# Autodesk Inventor assembly: Arm
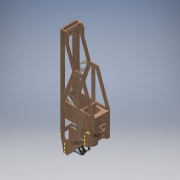
[picture p0: Inventor's stored thumbnail of the model, 180x180]
Saved by Autodesk Inventor 2019 (Build 230136000, 136)
## iProperties
Created: 2019-01-14
Part Number: Arm
Document SubType Name: Assembly
Designer: nxgam
Mass: 1682.66 g
Surface Area: 7952.13 cm^2
Volume: 1677.12 cm^3
Density: 1.0033 g/cm^3
Author: nxgam
## Documents named in this file (20)
- C:\Users\nxgam\Documents\CAD\Inventor\DiscoDraw\Arm.iam
- C:\Users\nxgam\Documents\CAD\Inventor\DiscoDraw\Arm.ipt
- C:\Users\nxgam\Documents\CAD\Inventor\DiscoDraw\Sled.iam
- C:\Users\nxgam\Documents\CAD\Inventor\DiscoDraw\ArmSpacer.ipt
- C:\Users\nxgam\Documents\CAD\Inventor\DiscoDraw\ArmSpacer3.ipt
- C:\Users\nxgam\Documents\CAD\Inventor\DiscoDraw\ArmSpacer6.ipt
- C:\Users\nxgam\Documents\CAD\Inventor\DiscoDraw\ArmTo.ipt
- C:\Users\nxgam\Documents\CAD\Inventor\DiscoDraw\ArmSide.ipt
- C:\Users\nxgam\Documents\CAD\Inventor\DiscoDraw\ArmMount.ipt
- C:\Users\nxgam\Documents\CAD\Inventor\DiscoDraw\MotorShelf.ipt
- C:\Users\nxgam\Documents\CAD\Inventor\DiscoDraw\EndPulleyMount.ipt
- C:\Users\nxgam\Documents\CAD\Inventor\DiscoDraw\ArmSideFrong2.ipt
- C:\Users\nxgam\Documents\CAD\Inventor\DiscoDraw\PiShelf.iam
- C:\Users\nxgam\Documents\CAD\Inventor\DiscoDraw\VerticalSupport.ipt
- C:\Users\nxgam\Documents\CAD\Inventor\DiscoDraw\LimitSwitch.ipt
- C:\Users\nxgam\Documents\CAD\Inventor\DiscoDraw\LimitSwitchMount.ipt
- C:\Users\nxgam\Documents\CAD\Inventor\DiscoDraw\BearingMount.ipt
- C:\Users\nxgam\Documents\CAD\Inventor\DiscoDraw\Imported\DC Motor\Motor assembly.ipt
- C:\Users\nxgam\Documents\CAD\Inventor\DiscoDraw\MotorMountDC.ipt
- C:\Users\nxgam\Documents\CAD\Inventor\DiscoDraw\MotorMountDCB.ipt
## Components (28 placed, 19 different names)
1. Arm:1 — Mate:1, Angle:1, Mate:4, Mate:5, Mate:6, Flush:3, Flush:4, Mate:7, Flush:12, Flush:13
2. Sled:1 [sub-assembly] — Mate:1, Angle:1, Flush:2, Flush:59
3. ArmSpacer:1 — Mate:3, Mate:5, Flush:1, Flush:4, Flush:10, Flush:11, Mate:8
4. ArmSpacer:2 — Mate:3, Mate:4, Flush:1, Flush:3
5. ArmSpacer3:1 — Flush:7, Mate:7, Flush:9
6. ArmSpacer3:3 — Flush:5, Flush:8
7. ArmSpacer6:1 — Flush:5, Flush:6, Flush:8, Flush:11
8. ArmSpacer6:2 — Flush:6, Flush:7, Flush:9, Flush:10
9. ArmTo:1 — Flush:12, Flush:13, Mate:8, Flush:28, Flush:29, Flush:31, Mate:20, Flush:54, Flush:57, Mate:31, Mate:32
10. ArmSide:1 — Flush:23, Flush:25, Flush:31, Flush:35, Flush:36, Flush:37, Mate:13, Mate:19, Flush:43, Flush:50, Mate:23, Flush:51, Mate:27, Mate:39
11. ArmSide:2 — Flush:26, Flush:27, Flush:28, Flush:29, Mate:15, Flush:46, Flush:49, Mate:21, Flush:50, Mate:24, Flush:55, Flush:56, Mate:30, Mate:37
12. ArmMount:1 — Flush:20, Flush:21, Flush:23, Flush:25, Flush:26, Flush:27, Mate:27, Mate:34, Mate:35, Angle:2
13. ArmMount:2 — Flush:20, Flush:21, Mate:28
14. VerticalSupport:2 — Flush:35, Flush:38, Mate:13
15. VerticalSupport:1 — Flush:36, Flush:37, Flush:38, Mate:15, Mate:36, Flush:61, Angle:3, Mate:42
16. EndPulleyMount:1 — Mate:19, Mate:20, Flush:53
17. ArmSideFrong2:1 — Flush:43, Flush:47, Flush:48, Mate:25, Flush:52, Mate:26, Flush:53, Flush:54, Mate:28
18. ArmSideFrong2:2 — Flush:46, Flush:47, Flush:48, Flush:49, Mate:21
19. PiShelf:1 [sub-assembly] — Flush:55, Flush:56, Mate:30
20. MotorShelf:1 — Mate:25, Flush:52, Mate:26
21. MotorShelf:2 — Mate:23, Mate:24, Flush:51
22. LimitSwitch:1 — Flush:57, Mate:31, Mate:33, Flush:58, Flush:60
23. LimitSwitchMount:1 — Mate:32, Mate:33, Flush:58
24. BearingMount:1 — Mate:34, Mate:35, Angle:2
25. Motor assembly:1 — Angle:3, Mate:41, Mate:42
26. MotorMountDC:1 — Mate:36, Flush:61, Mate:37, Mate:38, Flush:62
27. MotorMountDC:3
28. MotorMountDCB:1 — Mate:38, Flush:62, Mate:39, Mate:41
## Relationships (77: Flush 44, Mate 30, Angle 3)
- Mate:1: Arm:1 ↔ Sled:1
- Angle:1 (0 deg): Arm:1 ↔ Sled:1
- Mate:3: ArmSpacer:1 ↔ ArmSpacer:2
- Mate:4: Arm:1 ↔ ArmSpacer:2
- Mate:5: Arm:1 ↔ ArmSpacer:1
- Flush:1: ArmSpacer:1 ↔ ArmSpacer:2
- Flush:2 (-2.54 mm): Sled:1
- Mate:6: Arm:1
- Flush:3: Arm:1 ↔ ArmSpacer:2
- Flush:4: Arm:1 ↔ ArmSpacer:1
- Flush:5: ArmSpacer3:3 ↔ ArmSpacer6:1
- Flush:6: ArmSpacer6:1 ↔ ArmSpacer6:2
- Flush:7: ArmSpacer3:1 ↔ ArmSpacer6:2
- Mate:7: Arm:1 ↔ ArmSpacer3:1
- Flush:8: ArmSpacer3:3 ↔ ArmSpacer6:1
- Flush:9: ArmSpacer3:1 ↔ ArmSpacer6:2
- Flush:10: ArmSpacer:1 ↔ ArmSpacer6:2
- Flush:11: ArmSpacer:1 ↔ ArmSpacer6:1
- Flush:12: Arm:1 ↔ ArmTo:1
- Flush:13: Arm:1 ↔ ArmTo:1
- Mate:8: ArmSpacer:1 ↔ ArmTo:1
- Flush:20: ArmMount:1 ↔ ArmMount:2
- Flush:21: ArmMount:1 ↔ ArmMount:2
- Flush:23: ArmSide:1 ↔ ArmMount:1
- Flush:25: ArmSide:1 ↔ ArmMount:1
- Flush:26: ArmSide:2 ↔ ArmMount:1
- Flush:27: ArmSide:2 ↔ ArmMount:1
- Flush:28: ArmTo:1 ↔ ArmSide:2
- Flush:29: ArmTo:1 ↔ ArmSide:2
- Flush:31: ArmTo:1 ↔ ArmSide:1
- Flush:35: ArmSide:1 ↔ VerticalSupport:2
- Flush:36: ArmSide:1 ↔ VerticalSupport:1
- Flush:37: ArmSide:1 ↔ VerticalSupport:1
- Flush:38: VerticalSupport:2 ↔ VerticalSupport:1
- Mate:13: ArmSide:1 ↔ VerticalSupport:2
- Mate:15: ArmSide:2 ↔ VerticalSupport:1
- Mate:19: ArmSide:1 ↔ EndPulleyMount:1
- Mate:20 (20.32 mm): ArmTo:1 ↔ EndPulleyMount:1
- Flush:43: ArmSide:1 ↔ ArmSideFrong2:1
- Flush:46: ArmSide:2 ↔ ArmSideFrong2:2
- Flush:47: ArmSideFrong2:1 ↔ ArmSideFrong2:2
- Flush:48: ArmSideFrong2:1 ↔ ArmSideFrong2:2
- Flush:49: ArmSide:2 ↔ ArmSideFrong2:2
- Mate:21: ArmSide:2 ↔ ArmSideFrong2:2
- Flush:50: ArmSide:1 ↔ ArmSide:2
- Mate:23: ArmSide:1 ↔ MotorShelf:2
- Mate:24: ArmSide:2 ↔ MotorShelf:2
- Flush:51: ArmSide:1 ↔ MotorShelf:2
- Mate:25: ArmSideFrong2:1 ↔ MotorShelf:1
- Flush:52: ArmSideFrong2:1 ↔ MotorShelf:1
- Mate:26: ArmSideFrong2:1 ↔ MotorShelf:1
- Mate:27: ArmSide:1 ↔ ArmMount:1
- Flush:53: EndPulleyMount:1 ↔ ArmSideFrong2:1
- Flush:54: ArmTo:1 ↔ ArmSideFrong2:1
- Mate:28: ArmMount:2 ↔ ArmSideFrong2:1
- Flush:55: ArmSide:2 ↔ PiShelf:1
- Flush:56: ArmSide:2 ↔ PiShelf:1
- Flush:57: ArmTo:1 ↔ LimitSwitch:1
- Mate:30: ArmSide:2 ↔ PiShelf:1
- Mate:31: ArmTo:1 ↔ LimitSwitch:1
- Mate:32: ArmTo:1 ↔ LimitSwitchMount:1
- Mate:33: LimitSwitch:1 ↔ LimitSwitchMount:1
- Flush:58: LimitSwitch:1 ↔ LimitSwitchMount:1
- Flush:59 (-2.54 mm): Sled:1
- Flush:60: LimitSwitch:1
- Mate:34: ArmMount:1 ↔ BearingMount:1
- Mate:35: ArmMount:1 ↔ BearingMount:1
- Angle:2 (0 deg): ArmMount:1 ↔ BearingMount:1
- Mate:36: VerticalSupport:1 ↔ MotorMountDC:1
- Flush:61 (-12.7 mm): VerticalSupport:1 ↔ MotorMountDC:1
- Mate:37: ArmSide:2 ↔ MotorMountDC:1
- Mate:38: MotorMountDC:1 ↔ MotorMountDCB:1
- Flush:62: MotorMountDC:1 ↔ MotorMountDCB:1
- Mate:39: ArmSide:1 ↔ MotorMountDCB:1
- Angle:3 (90 deg): VerticalSupport:1 ↔ Motor assembly:1
- Mate:41: Motor assembly:1 ↔ MotorMountDCB:1
- Mate:42: VerticalSupport:1 ↔ Motor assembly:1
